# Autodesk Inventor assembly: Fermur
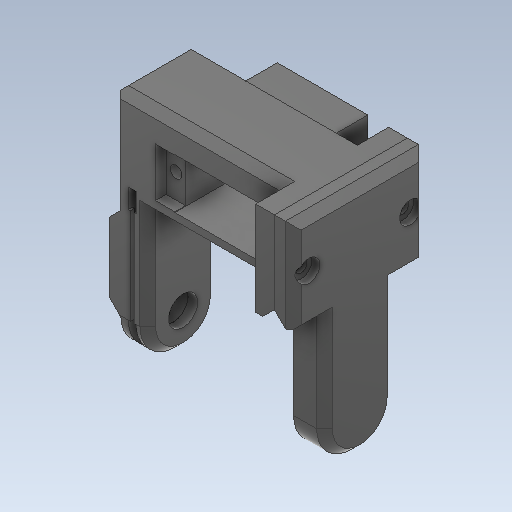
[picture p0: Inventor's stored thumbnail of the model, 512x512]
Saved by Autodesk Inventor 2020 (Build 240168000, 168)
## iProperties
Created: 2019-10-15
Part Number: Fermur
Document SubType Name: Assembly
Designer: Turing
Author: Turing
## Documents named in this file (4)
- D:\Hexapod Final Fucking Version 2\Fermur.iam
- D:\Hexapod Final Fucking Version 2\FermurSupport.ipt
- D:\Hexapod Final Fucking Version 2\FermurSupportSup.ipt
- D:\Hexapod Final Fucking Version 2\FemurSupportBot.ipt
## Components (3 placed, 3 different names)
1. FermurSupport:1 — Rigid:2, Rigid:3
2. FermurSupportSup:1 — Rigid:3
3. FemurSupportBot:1 — Rigid:2
## Relationships (2: WeldJoint 2)
- Rigid:2 [WeldJoint]: FermurSupport:1 ↔ FemurSupportBot:1
- Rigid:3 [WeldJoint]: FermurSupport:1 ↔ FermurSupportSup:1
